# Autodesk Inventor assembly: leg_press_assembly_aluminium_simulatible
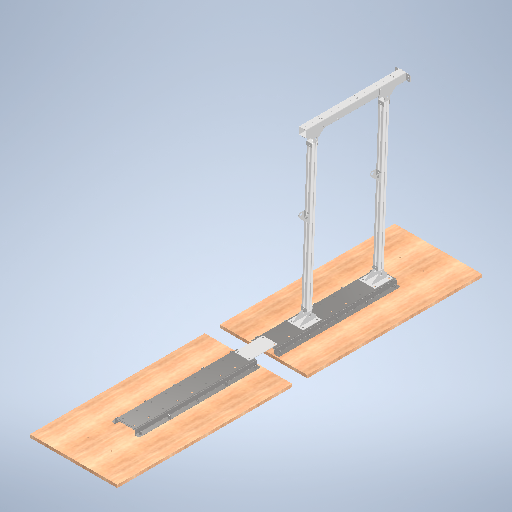
[picture p0: Inventor's stored thumbnail of the model, 512x512]
Saved by Autodesk Inventor 2025.2 (Build 292293000, 293)
## iProperties
Created: 2025-04-30
Part Number: leg_press_assembly_aluminium_simulatible
Document SubType Name: Assembly
Designer: Caspe
Author: Caspe
## Documents named in this file (8)
- C:\Users\Caspe\Documents\Semester 8\Project\Anomaly_Detection\Mechanical_Project\Inventor_project\leg_press_assembly_aluminium_simulatible.iam
- C:\Users\Caspe\Documents\Semester 8\Project\Anomaly_Detection\Mechanical_Project\Inventor_project\IMS-00-000_p&g.iam
- C:\Users\Caspe\Documents\Semester 8\Project\Anomaly_Detection\Mechanical_Project\Inventor_project\bottom_hinge.iam
- C:\Users\Caspe\Documents\Semester 8\Project\Anomaly_Detection\Mechanical_Project\Inventor_project\A_aluminium.iam
- C:\Users\Caspe\Documents\Semester 8\Project\Anomaly_Detection\Mechanical_Project\Inventor_project\Extender.ipt
- C:\Users\Caspe\Documents\Semester 8\Project\Anomaly_Detection\Mechanical_Project\Inventor_project\B_beam.iam
- C:\Users\Caspe\Documents\Semester 8\Project\Anomaly_Detection\Mechanical_Project\Inventor_project\A_B_hinge.ipt
- C:\Users\Caspe\Documents\Semester 8\Project\Anomaly_Detection\Mechanical_Project\Inventor_project\Leg_press_parameters.xlsx
## Components (12 placed, 6 different names)
1. IMS-00-000_p&g:1 [sub-assembly] — Insert:1, Insert:2, Insert:3, Insert:4, Insert:7, Insert:17
2. bottom_hinge:1 [sub-assembly] — Insert:1, Insert:2, Mate:1, Mate:2
3. A_aluminium:1 [sub-assembly] — Mate:1, Mate:2, Mate:5, Mate:7
4. IMS-00-000_p&g:2 [sub-assembly] — Insert:5, Insert:6
5. Extender:1 — Insert:3, Insert:4, Insert:5, Insert:6
6. bottom_hinge:2 [sub-assembly] — Insert:7, Insert:17
7. A_aluminium:2 [sub-assembly] — Mate:6
8. B_beam:1 [sub-assembly] — Insert:9, Insert:10, Insert:11, Insert:12, Insert:13, Insert:14, Insert:15, Insert:16
9. A_B_hinge:1 — Insert:9, Insert:10
10. A_B_hinge:2 — Insert:11, Insert:12, Mate:6
11. A_B_hinge:3 — Insert:15, Insert:16
12. A_B_hinge:4 — Insert:13, Insert:14, Mate:5, Mate:7
## Relationships (23: Insert 16, Mate 7)
- Insert:1: IMS-00-000_p&g:1 ↔ bottom_hinge:1
- Insert:2: IMS-00-000_p&g:1 ↔ bottom_hinge:1
- Mate:1: bottom_hinge:1 ↔ A_aluminium:1
- Mate:2 (1.5 mm): bottom_hinge:1 ↔ A_aluminium:1
- Insert:3: IMS-00-000_p&g:1 ↔ Extender:1
- Insert:4: IMS-00-000_p&g:1 ↔ Extender:1
- Insert:5: IMS-00-000_p&g:2 ↔ Extender:1
- Insert:6: IMS-00-000_p&g:2 ↔ Extender:1
- [Mate]: bottom_hinge:2 ↔ A_aluminium:2
- [Mate] (1.5 mm): bottom_hinge:2 ↔ A_aluminium:2
- Insert:7: IMS-00-000_p&g:1 ↔ bottom_hinge:2
- Insert:9: B_beam:1 ↔ A_B_hinge:1
- Insert:10: B_beam:1 ↔ A_B_hinge:1
- Insert:11: B_beam:1 ↔ A_B_hinge:2
- Insert:12: B_beam:1 ↔ A_B_hinge:2
- Insert:13: B_beam:1 ↔ A_B_hinge:4
- Insert:14: B_beam:1 ↔ A_B_hinge:4
- Insert:15: B_beam:1 ↔ A_B_hinge:3
- Insert:16: B_beam:1 ↔ A_B_hinge:3
- Mate:5: A_aluminium:1 ↔ A_B_hinge:4
- Mate:6: A_aluminium:2 ↔ A_B_hinge:2
- Mate:7 (3 mm): A_aluminium:1 ↔ A_B_hinge:4
- Insert:17: IMS-00-000_p&g:1 ↔ bottom_hinge:2
## Named parameters: A_length = 1000 mm, A_width = 40 mm, A_bend = 20 mm, A_connection_width = 40 mm, A_displacement = 500 mm, A_hole_height = 10 mm, A_hole_length = 40 mm, A_joint_diameter = 16 mm, A_height = 50 mm, A_B_spacing = 2 mm, A_joint_tolerance = 3 mm, l___________ = 0 mm, B_length = 700 mm, B_height = 50 mm, B_width = 50 mm, B_bend = 20 mm, B_connection_width = 40 mm, B_hole_height = 10 mm, B_hinge_holes_spacing = 50 mm, B_hole_length = 40 mm, l__________ = 0 mm, C_length = 400 mm, C_width = 20 mm, C_height = 330 mm, l_________ = 0 mm, rivet_diameter = 3.35 mm, rivet_displacement = 250 mm, plate_thickness = 1.5 mm, l________ = 0 mm, L_Piston_Top = 25 mm, L_Piston_Bottom = 21 mm, d8_d2 = 0 mm, d9_A_joint_tolerance = 3 mm, d10_d3 = 1.5 mm
